# Autodesk Inventor assembly: Assembly
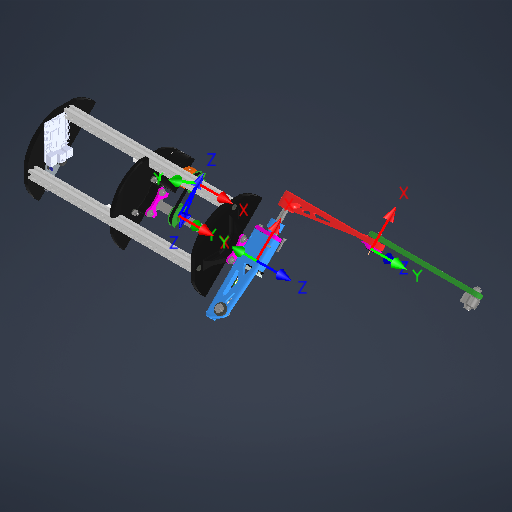
[picture p0: Inventor's stored thumbnail of the model, 512x512]
Saved by Autodesk Inventor 2027.1 (Build 311270010, 270A)
## iProperties
Created: 2026-10-15
Part Number: Assembly
Document SubType Name: Assembly
Designer: lucao
Author: lucao
## Documents named in this file (7)
- C:\Users\lucao\Desktop\RL-Rotary-Inverted-Double-Pendulum\CAD\Assembly.iam
- C:\Users\lucao\Desktop\RL-Rotary-Inverted-Double-Pendulum\CAD\AssemblyBase.iam
- C:\Users\lucao\Desktop\RL-Rotary-Inverted-Double-Pendulum\CAD\AssemblyMainAxis.iam
- C:\Users\lucao\Desktop\RL-Rotary-Inverted-Double-Pendulum\CAD\AssemblyPendulum1.iam
- C:\Users\lucao\Desktop\RL-Rotary-Inverted-Double-Pendulum\CAD\AssemblyPendulum2.iam
- C:\Users\lucao\Desktop\RL-Rotary-Inverted-Double-Pendulum\CAD\AssemblyDriveShaft.iam
- C:\Users\lucao\Desktop\RL-Rotary-Inverted-Double-Pendulum\CAD\timing_belt.ipt
## Components (6 placed, 6 different names)
1. AssemblyBase:1 [sub-assembly] — Mate:1, Mate:2, Mate:7, Mate:8, Flush:1, Mate:12
2. AssemblyMainAxis:1 [sub-assembly] — Mate:1, Mate:2, Mate:3, Mate:4, Mate:10, Rotation:1
3. AssemblyPendulum1:1 [sub-assembly] — Mate:3, Mate:4, Mate:5, Mate:6, Flush:1
4. AssemblyPendulum2:1 [sub-assembly] — Mate:5, Mate:6, Mate:12
5. AssemblyDriveShaft:1 [sub-assembly] — Mate:7, Mate:8, Mate:9, Mate:11, Rotation:1
6. timing_belt:1 — Mate:9, Mate:10, Mate:11
## Relationships (14: Mate 12, RelateRotation 1, Flush 1)
- Mate:1: AssemblyBase:1 ↔ AssemblyMainAxis:1
- Mate:2: AssemblyBase:1 ↔ AssemblyMainAxis:1
- Mate:3: AssemblyMainAxis:1 ↔ AssemblyPendulum1:1
- Mate:4: AssemblyMainAxis:1 ↔ AssemblyPendulum1:1
- Mate:5: AssemblyPendulum1:1 ↔ AssemblyPendulum2:1
- Mate:6: AssemblyPendulum1:1 ↔ AssemblyPendulum2:1
- Mate:7: AssemblyBase:1 ↔ AssemblyDriveShaft:1
- Mate:8: AssemblyBase:1 ↔ AssemblyDriveShaft:1
- Mate:9: AssemblyDriveShaft:1 ↔ timing_belt:1
- Mate:10: AssemblyMainAxis:1 ↔ timing_belt:1
- Mate:11: AssemblyDriveShaft:1 ↔ timing_belt:1
- Rotation:1 [RelateRotation] (1 ul): AssemblyMainAxis:1 ↔ AssemblyDriveShaft:1
- Flush:1: AssemblyBase:1 ↔ AssemblyPendulum1:1
- Mate:12: AssemblyBase:1 ↔ AssemblyPendulum2:1
## Named parameters: Simulation_Timeline = 0
